# Autodesk Inventor assembly: Bomba de agua
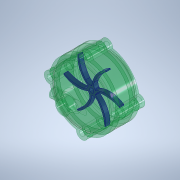
[picture p0: Inventor's stored thumbnail of the model, 180x180]
Saved by Autodesk Inventor 2020 (Build 240168000, 168)
## iProperties
Created: 2020-10-29
Part Number: Bomba de agua
Document SubType Name: Assembly
Designer: aaron
Author: aaron
## Documents named in this file (5)
- C:\Users\aaron\OneDrive\Escritorio\Proyecto\Bomba de agua\Bomba de agua.iam
- C:\Users\aaron\OneDrive\Escritorio\Proyecto\Bomba de agua\Central.ipt
- C:\Users\aaron\OneDrive\Escritorio\Proyecto\Bomba de agua\Propelas.ipt
- C:\Users\aaron\OneDrive\Escritorio\Proyecto\Bomba de agua\TapaE.ipt
- C:\Users\aaron\OneDrive\Escritorio\Proyecto\Bomba de agua\TapaS.ipt
## Components (4 placed, 4 different names)
1. Central:1 — Mate:1, Flush:1, Mate:2, Mate:3, Mate:4, Mate:5, Mate:6, Mate:7
2. Propelas:1 — Mate:1, Flush:1
3. TapaE:1 — Mate:2, Mate:3, Mate:4
4. TapaS:1 — Mate:5, Mate:6, Mate:7
## Relationships (8: Mate 7, Flush 1)
- Mate:1: Central:1 ↔ Propelas:1
- Flush:1 (1.5 mm): Central:1 ↔ Propelas:1
- Mate:2: Central:1 ↔ TapaE:1
- Mate:3: Central:1 ↔ TapaE:1
- Mate:4: Central:1 ↔ TapaE:1
- Mate:5: Central:1 ↔ TapaS:1
- Mate:6: Central:1 ↔ TapaS:1
- Mate:7: Central:1 ↔ TapaS:1
